# Autodesk Inventor assembly: ElevShortBackFrame
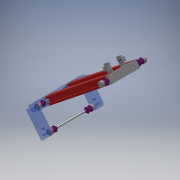
[picture p0: Inventor's stored thumbnail of the model, 180x180]
Saved by Autodesk Inventor 2019 (Build 230136000, 136)
## iProperties
Created: 2019-09-29
Part Number: ElevShortBackFrame
Document SubType Name: Weldment
Designer: james
Weld Material: Welded Aluminum-6061
Author: james
## Documents named in this file (9)
- F:\JimsDesign\Jims2020FTC\ElevShortBackFrame.iam
- F:\JimsDesign\Jims2020FTC\FullElevatorShart.iam
- F:\JimsDesign\Jims2020FTC\ElevBase.ipt
- F:\JimsDesign\Library\McMaster\SocketScrews\91251A201_BLACK-OXIDE ALLOY STEEL SOCKET HEAD SCREW.ipt
- F:\JimsDesign\Jims2020FTC\ElvatorEnd.iam
- F:\JimsDesign\Library\McMaster\Screws\91771A196_18-8 SS FLAT HEAD PHILLIPS MACHINE SCREW.ipt
- F:\JimsDesign\Jims2020FTC\SliderLeft.iam
- F:\JimsDesign\Jims2020FTC\SliderRight.iam
- F:\JimsDesign\Jims2020FTC\ShortBeamSplit.ipt
## Components (17 placed, 8 different names)
1. FullElevatorShart:1 [sub-assembly] — Mate:30, Mate:31
2. ElevBase:1 — Mate:11, Mate:12, Mate:13, Mate:14, Mate:15, Mate:16, Mate:17, Mate:18, Mate:19, Mate:20, Mate:33, Mate:36, Mate:43
3. FullElevatorShart:2 [sub-assembly] — Mate:11, Mate:12
4. 91251A201_BLACK-OXIDE ALLOY STEEL SOCKET HEAD SCREW:1 — Mate:16, Mate:17, Mate:42
5. 91251A201_BLACK-OXIDE ALLOY STEEL SOCKET HEAD SCREW:2 — Mate:15, Mate:19, Mate:35
6. 91251A201_BLACK-OXIDE ALLOY STEEL SOCKET HEAD SCREW:3 — Mate:14, Mate:20, Mate:34
7. 91251A201_BLACK-OXIDE ALLOY STEEL SOCKET HEAD SCREW:4 — Mate:13, Mate:18, Mate:41
8. ElvatorEnd:1 [sub-assembly] — Mate:30, Mate:31, Mate:32, Mate:44, Mate:45, Mate:48
9. FullElevatorShart:3 [sub-assembly] — Mate:32, Mate:33
10. 91771A196_18-8 SS FLAT HEAD PHILLIPS MACHINE SCREW:1 — Mate:37, Flush:2
11. 91771A196_18-8 SS FLAT HEAD PHILLIPS MACHINE SCREW:2 — Mate:38, Flush:1
12. 91771A196_18-8 SS FLAT HEAD PHILLIPS MACHINE SCREW:3 — Mate:40, Flush:3
13. 91771A196_18-8 SS FLAT HEAD PHILLIPS MACHINE SCREW:4 — Mate:39, Flush:4
14. SliderLeft:1 [sub-assembly] — Mate:46, Flush:5, Flush:6, Flush:7
15. SliderRight:1 [sub-assembly] — Mate:47, Flush:5, Flush:6, Mate:48
16. ShortBeamSplit:1 — Mate:34, Mate:35, Mate:36, Mate:39, Mate:40, Flush:3, Flush:4, Mate:44, Mate:45, Mate:47
17. ShortBeamSplit:2 — Mate:37, Mate:38, Flush:1, Flush:2, Mate:41, Mate:42, Mate:43, Mate:46, Flush:7
## Relationships (36: Mate 29, Flush 7)
- Mate:11: ElevBase:1 ↔ FullElevatorShart:2
- Mate:12: ElevBase:1 ↔ FullElevatorShart:2
- Mate:13: ElevBase:1 ↔ 91251A201_BLACK-OXIDE ALLOY STEEL SOCKET HEAD SCREW:4
- Mate:14: ElevBase:1 ↔ 91251A201_BLACK-OXIDE ALLOY STEEL SOCKET HEAD SCREW:3
- Mate:15: ElevBase:1 ↔ 91251A201_BLACK-OXIDE ALLOY STEEL SOCKET HEAD SCREW:2
- Mate:16: ElevBase:1 ↔ 91251A201_BLACK-OXIDE ALLOY STEEL SOCKET HEAD SCREW:1
- Mate:17: ElevBase:1 ↔ 91251A201_BLACK-OXIDE ALLOY STEEL SOCKET HEAD SCREW:1
- Mate:18: ElevBase:1 ↔ 91251A201_BLACK-OXIDE ALLOY STEEL SOCKET HEAD SCREW:4
- Mate:19: ElevBase:1 ↔ 91251A201_BLACK-OXIDE ALLOY STEEL SOCKET HEAD SCREW:2
- Mate:20: ElevBase:1 ↔ 91251A201_BLACK-OXIDE ALLOY STEEL SOCKET HEAD SCREW:3
- Mate:30: FullElevatorShart:1 ↔ ElvatorEnd:1
- Mate:31: FullElevatorShart:1 ↔ ElvatorEnd:1
- Mate:32: ElvatorEnd:1 ↔ FullElevatorShart:3
- Mate:33: ElevBase:1 ↔ FullElevatorShart:3
- Mate:34: 91251A201_BLACK-OXIDE ALLOY STEEL SOCKET HEAD SCREW:3 ↔ ShortBeamSplit:1
- Mate:35: 91251A201_BLACK-OXIDE ALLOY STEEL SOCKET HEAD SCREW:2 ↔ ShortBeamSplit:1
- Mate:36: ElevBase:1 ↔ ShortBeamSplit:1
- Mate:37: 91771A196_18-8 SS FLAT HEAD PHILLIPS MACHINE SCREW:1 ↔ ShortBeamSplit:2
- Mate:38: 91771A196_18-8 SS FLAT HEAD PHILLIPS MACHINE SCREW:2 ↔ ShortBeamSplit:2
- Flush:1: 91771A196_18-8 SS FLAT HEAD PHILLIPS MACHINE SCREW:2 ↔ ShortBeamSplit:2
- Flush:2: 91771A196_18-8 SS FLAT HEAD PHILLIPS MACHINE SCREW:1 ↔ ShortBeamSplit:2
- Mate:39: 91771A196_18-8 SS FLAT HEAD PHILLIPS MACHINE SCREW:4 ↔ ShortBeamSplit:1
- Mate:40: 91771A196_18-8 SS FLAT HEAD PHILLIPS MACHINE SCREW:3 ↔ ShortBeamSplit:1
- Flush:3: 91771A196_18-8 SS FLAT HEAD PHILLIPS MACHINE SCREW:3 ↔ ShortBeamSplit:1
- Flush:4: 91771A196_18-8 SS FLAT HEAD PHILLIPS MACHINE SCREW:4 ↔ ShortBeamSplit:1
- Mate:41: 91251A201_BLACK-OXIDE ALLOY STEEL SOCKET HEAD SCREW:4 ↔ ShortBeamSplit:2
- Mate:42: 91251A201_BLACK-OXIDE ALLOY STEEL SOCKET HEAD SCREW:1 ↔ ShortBeamSplit:2
- Mate:43: ElevBase:1 ↔ ShortBeamSplit:2
- Mate:44: ElvatorEnd:1 ↔ ShortBeamSplit:1
- Mate:45: ElvatorEnd:1 ↔ ShortBeamSplit:1
- Mate:46: SliderLeft:1 ↔ ShortBeamSplit:2
- Mate:47: SliderRight:1 ↔ ShortBeamSplit:1
- Flush:5: SliderLeft:1 ↔ SliderRight:1
- Flush:6: SliderLeft:1 ↔ SliderRight:1
- Mate:48: ElvatorEnd:1 ↔ SliderRight:1
- Flush:7: SliderLeft:1 ↔ ShortBeamSplit:2
